# Autodesk Inventor assembly: ASSEMBLY_Main
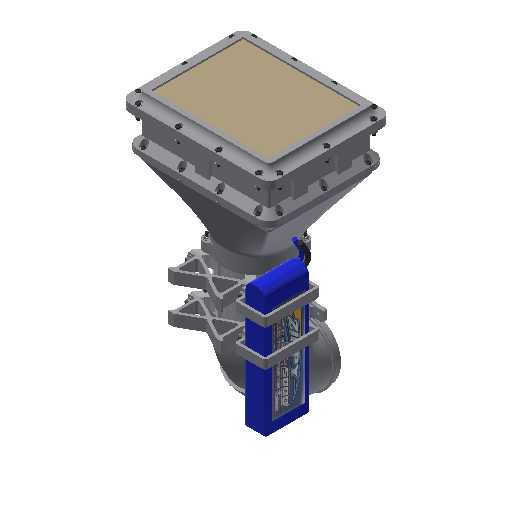
[picture p0: Inventor's stored thumbnail of the model, 512x512]
Saved by Autodesk Inventor 2025 (Build 290162010, 162A)
## iProperties
Created: 2020-03-28
Part Number: ASSEMBLY_Main
Document SubType Name: Assembly
Designer: Andrzej
Author: Andrzej
## Documents named in this file (25)
- D:\_ANDRZEJ_LACZEWSKI\_OTHER\MECH - Air Filtering Unit & Positive Pressure Suit (COVID-19)\MCAD\1_REV1\ASSEMBLY_MAIN_REVA\ASSEMBLY_Main.iam
- D:\_ANDRZEJ_LACZEWSKI\_OTHER\MECH - Air Filtering Unit & Positive Pressure Suit (COVID-19)\MCAD\1_REV1\ASSEMBLY_MAIN_REVA\3DP_PLA_Filter_stage.ipt
- D:\_ANDRZEJ_LACZEWSKI\_OTHER\MECH - Air Filtering Unit & Positive Pressure Suit (COVID-19)\MCAD\1_REV1\__COTS_PARTS\COTS_HP_BLC7000_Fan_Case.ipt
- D:\_ANDRZEJ_LACZEWSKI\_OTHER\MECH - Air Filtering Unit & Positive Pressure Suit (COVID-19)\MCAD\1_REV1\__COTS_PARTS\COTS_Zelmer_108x137mm_HEPA_filter.ipt
- D:\_ANDRZEJ_LACZEWSKI\_OTHER\MECH - Air Filtering Unit & Positive Pressure Suit (COVID-19)\MCAD\1_REV1\ASSEMBLY_MAIN_REVA\3DP_PLA_Filter_stage_to_turbine_adapter.ipt
- D:\_ANDRZEJ_LACZEWSKI\_OTHER\MECH - Air Filtering Unit & Positive Pressure Suit (COVID-19)\MCAD\1_REV1\ASSEMBLY_MAIN_REVA\3DP_PLA_Turbine_stand.ipt
- D:\_ANDRZEJ_LACZEWSKI\_OTHER\MECH - Air Filtering Unit & Positive Pressure Suit (COVID-19)\MCAD\1_REV1\ASSEMBLY_MAIN_REVA\3DP_PLA_Internal_filter_mesh.ipt
- D:\_ANDRZEJ_LACZEWSKI\_OTHER\MECH - Air Filtering Unit & Positive Pressure Suit (COVID-19)\MCAD\1_REV1\ASSEMBLY_MAIN_REVA\3DP_PLA_Front_filter_mount_hood.ipt
- D:\_ANDRZEJ_LACZEWSKI\_OTHER\MECH - Air Filtering Unit & Positive Pressure Suit (COVID-19)\MCAD\1_REV1\ASSEMBLY_MAIN_REVA\3DP_PLA_Front_filter_mount_hood_spacer.ipt
- D:\_ANDRZEJ_LACZEWSKI\_OTHER\MECH - Air Filtering Unit & Positive Pressure Suit (COVID-19)\MCAD\1_REV1\ASSEMBLY_MAIN_REVA\3DP_PLA_Front_filter_mesh.ipt
- D:\_ANDRZEJ_LACZEWSKI\_OTHER\MECH - Air Filtering Unit & Positive Pressure Suit (COVID-19)\MCAD\1_REV1\__COTS_PARTS\COTS_ZIPPY_Li-Po_Battery_5000mAh_3S.ipt
- D:\_ANDRZEJ_LACZEWSKI\_OTHER\MECH - Air Filtering Unit & Positive Pressure Suit (COVID-19)\MCAD\1_REV1\ASSEMBLY_MAIN_REVA\3DP_PLA_Battery_mount.ipt
- D:\_ANDRZEJ_LACZEWSKI\_OTHER\MECH - Air Filtering Unit & Positive Pressure Suit (COVID-19)\MCAD\1_REV1\ASSEMBLY_MAIN_REVA\3DP_PLA_Turbine_exhaust_bottom_part.ipt
- D:\_ANDRZEJ_LACZEWSKI\_OTHER\MECH - Air Filtering Unit & Positive Pressure Suit (COVID-19)\MCAD\1_REV1\ASSEMBLY_MAIN_REVA\3DP_PLA_Turbine_exhaust_top_part.ipt
- D:\_ANDRZEJ_LACZEWSKI\_OTHER\MECH - Air Filtering Unit & Positive Pressure Suit (COVID-19)\MCAD\1_REV1\ASSEMBLY_MAIN_REVA\3DP_PLA_Switch_&_handle_mount_plate.ipt
- D:\_ANDRZEJ_LACZEWSKI\_OTHER\MECH - Air Filtering Unit & Positive Pressure Suit (COVID-19)\MCAD\1_REV1\__CONTENT_CENTER_PARTS\en-US\DIN 125-2  A\DIN 125-2 - A 3,2A.ipt
- D:\_ANDRZEJ_LACZEWSKI\_OTHER\MECH - Air Filtering Unit & Positive Pressure Suit (COVID-19)\MCAD\1_REV1\__CONTENT_CENTER_PARTS\en-US\ISO 7380-1\ISO 7380-1 - M3 x 16.ipt
- D:\_ANDRZEJ_LACZEWSKI\_OTHER\MECH - Air Filtering Unit & Positive Pressure Suit (COVID-19)\MCAD\1_REV1\__CONTENT_CENTER_PARTS\en-US\DIN 934\DIN 934 - M3 x 0,5.ipt
- D:\_ANDRZEJ_LACZEWSKI\_OTHER\MECH - Air Filtering Unit & Positive Pressure Suit (COVID-19)\MCAD\1_REV1\__CONTENT_CENTER_PARTS\en-US\ISO 7380-1\ISO 7380-1 - M3 x 10.ipt
- D:\_ANDRZEJ_LACZEWSKI\_OTHER\MECH - Air Filtering Unit & Positive Pressure Suit (COVID-19)\MCAD\1_REV1\__CONTENT_CENTER_PARTS\en-US\DIN 125-2  A\DIN 125-2 - A 4,3A.ipt
- D:\_ANDRZEJ_LACZEWSKI\_OTHER\MECH - Air Filtering Unit & Positive Pressure Suit (COVID-19)\MCAD\1_REV1\__CONTENT_CENTER_PARTS\en-US\ISO 7380-1\ISO 7380-1 - M4 x 12.ipt
- D:\_ANDRZEJ_LACZEWSKI\_OTHER\MECH - Air Filtering Unit & Positive Pressure Suit (COVID-19)\MCAD\1_REV1\__CONTENT_CENTER_PARTS\en-US\DIN 934\DIN 934 - M4 x 0,7.ipt
- D:\_ANDRZEJ_LACZEWSKI\_OTHER\MECH - Air Filtering Unit & Positive Pressure Suit (COVID-19)\MCAD\1_REV1\__CONTENT_CENTER_PARTS\en-US\ISO 7380-1\ISO 7380-1 - M3 x 30.ipt
- D:\_ANDRZEJ_LACZEWSKI\_OTHER\MECH - Air Filtering Unit & Positive Pressure Suit (COVID-19)\MCAD\1_REV1\__CONTENT_CENTER_PARTS\en-US\ISO 7380-1\ISO 7380-1 - M4 x 20.ipt
- D:\_ANDRZEJ_LACZEWSKI\_OTHER\MECH - Air Filtering Unit & Positive Pressure Suit (COVID-19)\MCAD\1_REV1\__CONTENT_CENTER_PARTS\en-US\ISO 7380-1\ISO 7380-1 - M4 x 16.ipt
## Components (164 placed, 24 different names)
1. 3DP_PLA_Filter_stage:1 — Mate:1, Mate:2, Mate:3, Mate:4, Flush:1, Flush:2, Mate:13, Mate:14, Mate:16, Flush:3, Flush:4, Mate:82, Mate:84, Mate:86, Mate:88, Mate:90, Mate:92, Mate:94, Mate:96, Mate:98, Mate:100, Mate:102, Mate:104, Mate:106, Mate:108, Mate:109, Mate:110, Mate:111, Mate:112, Mate:113, Mate:114, Mate:115, Mate:116, Mate:117, Mate:118, Mate:119, Mate:120, Mate:121, Mate:122, Mate:123, Mate:124, Mate:125, Mate:126, Mate:127, Mate:128, Mate:129, Mate:130, Mate:131, Mate:132, Mate:133, Mate:134, Mate:135, Mate:136, Mate:137, Mate:139, Mate:141, Mate:143, Mate:145, Mate:147, Mate:149, Mate:151, Mate:153, Mate:155, Mate:157, Mate:159, Mate:161, Mate:163
2. COTS_HP_BLC7000_Fan_Case:1 — Mate:5, Mate:6, Mate:9, Mate:10, Mate:11, Mate:21, Mate:22, Mate:26, Mate:27, Mate:28, Mate:29, Mate:30, Mate:31, Mate:32, Mate:33, Mate:48, Mate:49, Mate:50, Mate:165, Mate:166, Mate:167, Mate:168, Mate:169, Mate:171, Mate:173, Mate:174, Mate:175, Mate:176, Mate:177, Mate:179, Mate:181, Mate:182, Mate:183, Mate:184, Mate:185, Mate:187
3. COTS_Zelmer_108x137mm_HEPA_filter:1 — Mate:1, Mate:2, Mate:3, Mate:23
4. 3DP_PLA_Filter_stage_to_turbine_adapter:1 — Mate:4, Flush:1, Flush:2, Mate:5, Mate:6, Mate:9, Mate:12, Mate:138, Mate:140, Mate:142, Mate:144, Mate:146, Mate:148, Mate:150, Mate:152, Mate:154, Mate:156, Mate:158, Mate:160, Mate:162, Mate:164, Mate:178, Mate:180
5. 3DP_PLA_Turbine_stand:1 — Mate:10, Mate:11, Mate:26
6. 3DP_PLA_Internal_filter_mesh:1 — Mate:12, Mate:13, Mate:14
7. 3DP_PLA_Front_filter_mount_hood:1 — Mate:17, Flush:5, Flush:6, Mate:44, Mate:45, Mate:53, Mate:54, Mate:55, Mate:56, Mate:57, Mate:58, Mate:59, Mate:60, Mate:61, Mate:62, Mate:63, Mate:64, Mate:65, Mate:66, Mate:67, Mate:68, Mate:69, Mate:70, Mate:71, Mate:72, Mate:73, Mate:74, Mate:75, Mate:76, Mate:77, Mate:78, Mate:79, Mate:80, Mate:81, Mate:83, Mate:85, Mate:87, Mate:89, Mate:91, Mate:93, Mate:95, Mate:97, Mate:99, Mate:101, Mate:103, Mate:105, Mate:107
8. 3DP_PLA_Front_filter_mount_hood_spacer:1 — Mate:16, Flush:3, Flush:4, Mate:17, Flush:5, Flush:6
9. 3DP_PLA_Turbine_stand:2 — Mate:21, Mate:22, Mate:27, Mate:170, Mate:172
10. 3DP_PLA_Front_filter_mesh:1 — Mate:23, Mate:44, Mate:45
11. COTS_ZIPPY_Li-Po_Battery_5000mAh_3S:1 — Mate:34, Mate:35
12. 3DP_PLA_Battery_mount:1 — Mate:28, Mate:29, Mate:30, Mate:34, Mate:35, Mate:189, Mate:190, Mate:192, Mate:193, Mate:194, Mate:196
13. 3DP_PLA_Battery_mount:2 — Mate:31, Mate:32, Mate:33, Mate:191, Mate:195
14. 3DP_PLA_Turbine_exhaust_bottom_part:1 — Mate:46, Mate:47, Tangent:1, Mate:48, Mate:49, Mate:50, Mate:51, Mate:52, Mate:186, Mate:188
15. 3DP_PLA_Turbine_exhaust_top_part:1 — Mate:46, Mate:47, Tangent:1
16. 3DP_PLA_Switch_&_handle_mount_plate:1 — Mate:51, Mate:52, Mate:197, Mate:198, Mate:199, Mate:200
17. ISO 7380-1 M4 x 16:2 — Insert:74
18. DIN 125-2 A A 4,3:10 — Mate:199, Mate:200, Insert:74
19. ISO 7380-1 M4 x 16:1 — Insert:73
20. DIN 125-2 A A 4,3:9 — Mate:197, Mate:198, Insert:73
21. DIN 934 - replaced by DIN EN 24032/28673/28674 M4:4 — Insert:72
22. DIN 125-2 A A 4,3:8 — Mate:195, Mate:196, Insert:72
23. ISO 7380-1 M4 x 20:2 — Insert:70
24. DIN 125-2 A A 4,3:7 — Mate:191, Mate:192, Insert:70
25. DIN 934 - replaced by DIN EN 24032/28673/28674 M4:3 — Insert:71
26. DIN 125-2 A A 4,3:6 — Mate:193, Mate:194, Insert:71
27. ISO 7380-1 M4 x 20:1 — Insert:69
28. DIN 125-2 A A 4,3:5 — Mate:189, Mate:190, Insert:69
29. DIN 934 - replaced by DIN EN 24032/28673/28674 M3:32 — Insert:68
30. DIN 125-2 A A 3,2:64 — Mate:187, Mate:188, Insert:68
31. ISO 7380-1 M3 x 30:4 — Insert:66
32. DIN 125-2 A A 3,2:63 — Mate:183, Mate:184, Insert:66
33. DIN 934 - replaced by DIN EN 24032/28673/28674 M3:31 — Insert:67
34. DIN 125-2 A A 3,2:62 — Mate:185, Mate:186, Insert:67
35. ISO 7380-1 M3 x 30:3 — Insert:65
36. DIN 125-2 A A 3,2:61 — Mate:181, Mate:182, Insert:65
37. DIN 934 - replaced by DIN EN 24032/28673/28674 M3:30 — Insert:64
38. DIN 125-2 A A 3,2:60 — Mate:179, Mate:180, Insert:64
39. ISO 7380-1 M3 x 30:2 — Insert:62
40. DIN 125-2 A A 3,2:59 — Mate:175, Mate:176, Insert:62
41. DIN 934 - replaced by DIN EN 24032/28673/28674 M3:29 — Insert:63
42. DIN 125-2 A A 3,2:58 — Mate:177, Mate:178, Insert:63
43. ISO 7380-1 M3 x 30:1 — Insert:61
44. DIN 125-2 A A 3,2:57 — Mate:173, Mate:174, Insert:61
45. DIN 934 - replaced by DIN EN 24032/28673/28674 M4:2 — Insert:60
46. DIN 125-2 A A 4,3:4 — Mate:171, Mate:172, Insert:60
47. ISO 7380-1 M4 x 12:2 — Insert:58
48. DIN 125-2 A A 4,3:3 — Mate:167, Mate:168, Insert:58
49. DIN 934 - replaced by DIN EN 24032/28673/28674 M4:1 — Insert:59
50. DIN 125-2 A A 4,3:2 — Mate:169, Mate:170, Insert:59
51. ISO 7380-1 M4 x 12:1 — Insert:57
52. DIN 125-2 A A 4,3:1 — Mate:165, Mate:166, Insert:57
53. DIN 934 - replaced by DIN EN 24032/28673/28674 M3:28 — Insert:56
54. DIN 934 - replaced by DIN EN 24032/28673/28674 M3:27 — Insert:55
55. DIN 934 - replaced by DIN EN 24032/28673/28674 M3:26 — Insert:54
56. DIN 934 - replaced by DIN EN 24032/28673/28674 M3:25 — Insert:53
57. DIN 934 - replaced by DIN EN 24032/28673/28674 M3:24 — Insert:52
58. DIN 934 - replaced by DIN EN 24032/28673/28674 M3:23 — Insert:51
59. DIN 934 - replaced by DIN EN 24032/28673/28674 M3:22 — Insert:50
60. DIN 934 - replaced by DIN EN 24032/28673/28674 M3:21 — Insert:49
61. DIN 934 - replaced by DIN EN 24032/28673/28674 M3:20 — Insert:48
62. DIN 934 - replaced by DIN EN 24032/28673/28674 M3:19 — Insert:47
63. DIN 934 - replaced by DIN EN 24032/28673/28674 M3:18 — Insert:46
64. DIN 934 - replaced by DIN EN 24032/28673/28674 M3:17 — Insert:45
65. DIN 934 - replaced by DIN EN 24032/28673/28674 M3:16 — Insert:44
66. DIN 125-2 A A 3,2:56 — Mate:163, Mate:164, Insert:56
67. DIN 125-2 A A 3,2:55 — Mate:161, Mate:162, Insert:55
68. DIN 125-2 A A 3,2:54 — Mate:159, Mate:160, Insert:54
69. DIN 125-2 A A 3,2:53 — Mate:157, Mate:158, Insert:53
70. DIN 125-2 A A 3,2:52 — Mate:155, Mate:156, Insert:52
71. DIN 125-2 A A 3,2:51 — Mate:153, Mate:154, Insert:51
72. DIN 125-2 A A 3,2:50 — Mate:151, Mate:152, Insert:50
73. DIN 125-2 A A 3,2:49 — Mate:149, Mate:150, Insert:49
74. DIN 125-2 A A 3,2:48 — Mate:147, Mate:148, Insert:48
75. DIN 125-2 A A 3,2:47 — Mate:145, Mate:146, Insert:47
76. DIN 125-2 A A 3,2:46 — Mate:143, Mate:144, Insert:46
77. DIN 125-2 A A 3,2:45 — Mate:141, Mate:142, Insert:45
78. DIN 125-2 A A 3,2:44 — Mate:139, Mate:140, Insert:44
79. ISO 7380-1 M3 x 10:14 — Insert:42
80. ISO 7380-1 M3 x 10:13 — Insert:41
81. ISO 7380-1 M3 x 10:12 — Insert:40
82. ISO 7380-1 M3 x 10:11 — Insert:39
83. ISO 7380-1 M3 x 10:10 — Insert:38
84. ISO 7380-1 M3 x 10:9 — Insert:37
85. ISO 7380-1 M3 x 10:8 — Insert:36
86. ISO 7380-1 M3 x 10:7 — Insert:35
87. ISO 7380-1 M3 x 10:6 — Insert:34
88. ISO 7380-1 M3 x 10:5 — Insert:33
89. ISO 7380-1 M3 x 10:4 — Insert:32
90. ISO 7380-1 M3 x 10:3 — Insert:31
91. ISO 7380-1 M3 x 10:2 — Insert:30
92. DIN 125-2 A A 3,2:43 — Mate:135, Mate:136, Insert:42
93. DIN 125-2 A A 3,2:42 — Mate:133, Mate:134, Insert:41
94. DIN 125-2 A A 3,2:41 — Mate:131, Mate:132, Insert:40
95. DIN 125-2 A A 3,2:40 — Mate:129, Mate:130, Insert:39
96. DIN 125-2 A A 3,2:39 — Mate:127, Mate:128, Insert:38
97. DIN 125-2 A A 3,2:38 — Mate:125, Mate:126, Insert:37
98. DIN 125-2 A A 3,2:37 — Mate:123, Mate:124, Insert:36
99. DIN 125-2 A A 3,2:36 — Mate:121, Mate:122, Insert:35
100. DIN 125-2 A A 3,2:35 — Mate:119, Mate:120, Insert:34
101. DIN 125-2 A A 3,2:34 — Mate:117, Mate:118, Insert:33
102. DIN 125-2 A A 3,2:33 — Mate:115, Mate:116, Insert:32
103. DIN 125-2 A A 3,2:32 — Mate:113, Mate:114, Insert:31
104. DIN 125-2 A A 3,2:31 — Mate:111, Mate:112, Insert:30
105. DIN 934 - replaced by DIN EN 24032/28673/28674 M3:15 — Insert:43
106. DIN 125-2 A A 3,2:30 — Mate:137, Mate:138, Insert:43
107. ISO 7380-1 M3 x 10:1 — Insert:29
108. DIN 125-2 A A 3,2:29 — Mate:109, Mate:110, Insert:29
109. DIN 934 - replaced by DIN EN 24032/28673/28674 M3:14 — Insert:28
110. DIN 934 - replaced by DIN EN 24032/28673/28674 M3:13 — Insert:27
111. DIN 934 - replaced by DIN EN 24032/28673/28674 M3:12 — Insert:26
112. DIN 934 - replaced by DIN EN 24032/28673/28674 M3:11 — Insert:25
113. DIN 934 - replaced by DIN EN 24032/28673/28674 M3:10 — Insert:24
114. DIN 934 - replaced by DIN EN 24032/28673/28674 M3:9 — Insert:23
115. DIN 934 - replaced by DIN EN 24032/28673/28674 M3:8 — Insert:22
116. DIN 934 - replaced by DIN EN 24032/28673/28674 M3:7 — Insert:21
117. DIN 934 - replaced by DIN EN 24032/28673/28674 M3:6 — Insert:20
118. DIN 934 - replaced by DIN EN 24032/28673/28674 M3:5 — Insert:19
119. DIN 934 - replaced by DIN EN 24032/28673/28674 M3:4 — Insert:18
120. DIN 934 - replaced by DIN EN 24032/28673/28674 M3:3 — Insert:17
121. DIN 934 - replaced by DIN EN 24032/28673/28674 M3:2 — Insert:16
122. DIN 125-2 A A 3,2:28 — Mate:107, Mate:108, Insert:28
123. DIN 125-2 A A 3,2:27 — Mate:105, Mate:106, Insert:27
124. DIN 125-2 A A 3,2:26 — Mate:103, Mate:104, Insert:26
125. DIN 125-2 A A 3,2:25 — Mate:101, Mate:102, Insert:25
126. DIN 125-2 A A 3,2:24 — Mate:99, Mate:100, Insert:24
127. DIN 125-2 A A 3,2:23 — Mate:97, Mate:98, Insert:23
128. DIN 125-2 A A 3,2:22 — Mate:95, Mate:96, Insert:22
129. DIN 125-2 A A 3,2:21 — Mate:93, Mate:94, Insert:21
130. DIN 125-2 A A 3,2:20 — Mate:91, Mate:92, Insert:20
131. DIN 125-2 A A 3,2:19 — Mate:89, Mate:90, Insert:19
132. DIN 125-2 A A 3,2:18 — Mate:87, Mate:88, Insert:18
133. DIN 125-2 A A 3,2:17 — Mate:85, Mate:86, Insert:17
134. DIN 125-2 A A 3,2:16 — Mate:83, Mate:84, Insert:16
135. ISO 7380-1 M3 x 16:14 — Insert:14
136. ISO 7380-1 M3 x 16:13 — Insert:13
137. ISO 7380-1 M3 x 16:12 — Insert:12
138. ISO 7380-1 M3 x 16:11 — Insert:11
139. ISO 7380-1 M3 x 16:10 — Insert:10
140. ISO 7380-1 M3 x 16:9 — Insert:9
141. ISO 7380-1 M3 x 16:8 — Insert:8
142. ISO 7380-1 M3 x 16:7 — Insert:7
143. ISO 7380-1 M3 x 16:6 — Insert:6
144. ISO 7380-1 M3 x 16:5 — Insert:5
145. ISO 7380-1 M3 x 16:4 — Insert:4
146. ISO 7380-1 M3 x 16:3 — Insert:3
147. ISO 7380-1 M3 x 16:2 — Insert:2
148. DIN 125-2 A A 3,2:15 — Mate:79, Mate:80, Insert:14
149. DIN 125-2 A A 3,2:14 — Mate:77, Mate:78, Insert:13
150. DIN 125-2 A A 3,2:13 — Mate:75, Mate:76, Insert:12
151. DIN 125-2 A A 3,2:12 — Mate:73, Mate:74, Insert:11
152. DIN 125-2 A A 3,2:11 — Mate:71, Mate:72, Insert:10
153. DIN 125-2 A A 3,2:10 — Mate:69, Mate:70, Insert:9
154. DIN 125-2 A A 3,2:9 — Mate:67, Mate:68, Insert:8
155. DIN 125-2 A A 3,2:8 — Mate:65, Mate:66, Insert:7
156. DIN 125-2 A A 3,2:7 — Mate:63, Mate:64, Insert:6
157. DIN 125-2 A A 3,2:6 — Mate:61, Mate:62, Insert:5
158. DIN 125-2 A A 3,2:5 — Mate:59, Mate:60, Insert:4
159. DIN 125-2 A A 3,2:4 — Mate:57, Mate:58, Insert:3
160. DIN 125-2 A A 3,2:3 — Mate:55, Mate:56, Insert:2
161. DIN 934 - replaced by DIN EN 24032/28673/28674 M3:1 — Insert:15
162. DIN 125-2 A A 3,2:2 — Mate:81, Mate:82, Insert:15
163. ISO 7380-1 M3 x 16:1 — Insert:1
164. DIN 125-2 A A 3,2:1 — Mate:53, Mate:54, Insert:1
## Relationships (265: Mate 184, Insert 74, Flush 6, Tangent 1)
- Mate:1: 3DP_PLA_Filter_stage:1 ↔ COTS_Zelmer_108x137mm_HEPA_filter:1
- Mate:2 (1 mm): 3DP_PLA_Filter_stage:1 ↔ COTS_Zelmer_108x137mm_HEPA_filter:1
- Mate:3 (1 mm): 3DP_PLA_Filter_stage:1 ↔ COTS_Zelmer_108x137mm_HEPA_filter:1
- Mate:4: 3DP_PLA_Filter_stage:1 ↔ 3DP_PLA_Filter_stage_to_turbine_adapter:1
- Flush:1: 3DP_PLA_Filter_stage:1 ↔ 3DP_PLA_Filter_stage_to_turbine_adapter:1
- Flush:2: 3DP_PLA_Filter_stage:1 ↔ 3DP_PLA_Filter_stage_to_turbine_adapter:1
- Mate:5: COTS_HP_BLC7000_Fan_Case:1 ↔ 3DP_PLA_Filter_stage_to_turbine_adapter:1
- Mate:6: COTS_HP_BLC7000_Fan_Case:1 ↔ 3DP_PLA_Filter_stage_to_turbine_adapter:1
- Mate:9: COTS_HP_BLC7000_Fan_Case:1 ↔ 3DP_PLA_Filter_stage_to_turbine_adapter:1
- Mate:10: COTS_HP_BLC7000_Fan_Case:1 ↔ 3DP_PLA_Turbine_stand:1
- Mate:11: COTS_HP_BLC7000_Fan_Case:1 ↔ 3DP_PLA_Turbine_stand:1
- Mate:12: 3DP_PLA_Filter_stage_to_turbine_adapter:1 ↔ 3DP_PLA_Internal_filter_mesh:1
- Mate:13 (0.5 mm): 3DP_PLA_Filter_stage:1 ↔ 3DP_PLA_Internal_filter_mesh:1
- Mate:14 (0.5 mm): 3DP_PLA_Filter_stage:1 ↔ 3DP_PLA_Internal_filter_mesh:1
- Mate:16: 3DP_PLA_Filter_stage:1 ↔ 3DP_PLA_Front_filter_mount_hood_spacer:1
- Flush:3: 3DP_PLA_Filter_stage:1 ↔ 3DP_PLA_Front_filter_mount_hood_spacer:1
- Flush:4: 3DP_PLA_Filter_stage:1 ↔ 3DP_PLA_Front_filter_mount_hood_spacer:1
- Mate:17: 3DP_PLA_Front_filter_mount_hood:1 ↔ 3DP_PLA_Front_filter_mount_hood_spacer:1
- Flush:5: 3DP_PLA_Front_filter_mount_hood:1 ↔ 3DP_PLA_Front_filter_mount_hood_spacer:1
- Flush:6: 3DP_PLA_Front_filter_mount_hood:1 ↔ 3DP_PLA_Front_filter_mount_hood_spacer:1
- Mate:21: COTS_HP_BLC7000_Fan_Case:1 ↔ 3DP_PLA_Turbine_stand:2
- Mate:22: COTS_HP_BLC7000_Fan_Case:1 ↔ 3DP_PLA_Turbine_stand:2
- Mate:23 (3 mm): COTS_Zelmer_108x137mm_HEPA_filter:1 ↔ 3DP_PLA_Front_filter_mesh:1
- Mate:26: COTS_HP_BLC7000_Fan_Case:1 ↔ 3DP_PLA_Turbine_stand:1
- Mate:27: COTS_HP_BLC7000_Fan_Case:1 ↔ 3DP_PLA_Turbine_stand:2
- Mate:28 (0.1 mm): COTS_HP_BLC7000_Fan_Case:1 ↔ 3DP_PLA_Battery_mount:1
- Mate:29: COTS_HP_BLC7000_Fan_Case:1 ↔ 3DP_PLA_Battery_mount:1
- Mate:30: COTS_HP_BLC7000_Fan_Case:1 ↔ 3DP_PLA_Battery_mount:1
- Mate:31: COTS_HP_BLC7000_Fan_Case:1 ↔ 3DP_PLA_Battery_mount:2
- Mate:32 (0.1 mm): COTS_HP_BLC7000_Fan_Case:1 ↔ 3DP_PLA_Battery_mount:2
- Mate:33: COTS_HP_BLC7000_Fan_Case:1 ↔ 3DP_PLA_Battery_mount:2
- Mate:34 (3 mm): COTS_ZIPPY_Li-Po_Battery_5000mAh_3S:1 ↔ 3DP_PLA_Battery_mount:1
- Mate:35 (3 mm): COTS_ZIPPY_Li-Po_Battery_5000mAh_3S:1 ↔ 3DP_PLA_Battery_mount:1
- Mate:44 (0.5 mm): 3DP_PLA_Front_filter_mount_hood:1 ↔ 3DP_PLA_Front_filter_mesh:1
- Mate:45 (0.5 mm): 3DP_PLA_Front_filter_mount_hood:1 ↔ 3DP_PLA_Front_filter_mesh:1
- Mate:46: 3DP_PLA_Turbine_exhaust_bottom_part:1 ↔ 3DP_PLA_Turbine_exhaust_top_part:1
- Mate:47: 3DP_PLA_Turbine_exhaust_bottom_part:1 ↔ 3DP_PLA_Turbine_exhaust_top_part:1
- Tangent:1: 3DP_PLA_Turbine_exhaust_bottom_part:1 ↔ 3DP_PLA_Turbine_exhaust_top_part:1
- Mate:48: COTS_HP_BLC7000_Fan_Case:1 ↔ 3DP_PLA_Turbine_exhaust_bottom_part:1
- Mate:49: COTS_HP_BLC7000_Fan_Case:1 ↔ 3DP_PLA_Turbine_exhaust_bottom_part:1
- Mate:50: COTS_HP_BLC7000_Fan_Case:1 ↔ 3DP_PLA_Turbine_exhaust_bottom_part:1
- Mate:51: 3DP_PLA_Turbine_exhaust_bottom_part:1 ↔ 3DP_PLA_Switch_&_handle_mount_plate:1
- Mate:52: 3DP_PLA_Turbine_exhaust_bottom_part:1 ↔ 3DP_PLA_Switch_&_handle_mount_plate:1
- Mate:53: 3DP_PLA_Front_filter_mount_hood:1 ↔ DIN 125-2 A A 3,2:1
- Mate:54: 3DP_PLA_Front_filter_mount_hood:1 ↔ DIN 125-2 A A 3,2:1
- Mate:55: 3DP_PLA_Front_filter_mount_hood:1 ↔ DIN 125-2 A A 3,2:3
- Mate:56: 3DP_PLA_Front_filter_mount_hood:1 ↔ DIN 125-2 A A 3,2:3
- Mate:57: 3DP_PLA_Front_filter_mount_hood:1 ↔ DIN 125-2 A A 3,2:4
- Mate:58: 3DP_PLA_Front_filter_mount_hood:1 ↔ DIN 125-2 A A 3,2:4
- Mate:59: 3DP_PLA_Front_filter_mount_hood:1 ↔ DIN 125-2 A A 3,2:5
- Mate:60: 3DP_PLA_Front_filter_mount_hood:1 ↔ DIN 125-2 A A 3,2:5
- Mate:61: 3DP_PLA_Front_filter_mount_hood:1 ↔ DIN 125-2 A A 3,2:6
- Mate:62: 3DP_PLA_Front_filter_mount_hood:1 ↔ DIN 125-2 A A 3,2:6
- Mate:63: 3DP_PLA_Front_filter_mount_hood:1 ↔ DIN 125-2 A A 3,2:7
- Mate:64: 3DP_PLA_Front_filter_mount_hood:1 ↔ DIN 125-2 A A 3,2:7
- Mate:65: 3DP_PLA_Front_filter_mount_hood:1 ↔ DIN 125-2 A A 3,2:8
- Mate:66: 3DP_PLA_Front_filter_mount_hood:1 ↔ DIN 125-2 A A 3,2:8
- Mate:67: 3DP_PLA_Front_filter_mount_hood:1 ↔ DIN 125-2 A A 3,2:9
- Mate:68: 3DP_PLA_Front_filter_mount_hood:1 ↔ DIN 125-2 A A 3,2:9
- Mate:69: 3DP_PLA_Front_filter_mount_hood:1 ↔ DIN 125-2 A A 3,2:10
- Mate:70: 3DP_PLA_Front_filter_mount_hood:1 ↔ DIN 125-2 A A 3,2:10
- Mate:71: 3DP_PLA_Front_filter_mount_hood:1 ↔ DIN 125-2 A A 3,2:11
- Mate:72: 3DP_PLA_Front_filter_mount_hood:1 ↔ DIN 125-2 A A 3,2:11
- Mate:73: 3DP_PLA_Front_filter_mount_hood:1 ↔ DIN 125-2 A A 3,2:12
- Mate:74: 3DP_PLA_Front_filter_mount_hood:1 ↔ DIN 125-2 A A 3,2:12
- Mate:75: 3DP_PLA_Front_filter_mount_hood:1 ↔ DIN 125-2 A A 3,2:13
- Mate:76: 3DP_PLA_Front_filter_mount_hood:1 ↔ DIN 125-2 A A 3,2:13
- Mate:77: 3DP_PLA_Front_filter_mount_hood:1 ↔ DIN 125-2 A A 3,2:14
- Mate:78: 3DP_PLA_Front_filter_mount_hood:1 ↔ DIN 125-2 A A 3,2:14
- Mate:79: 3DP_PLA_Front_filter_mount_hood:1 ↔ DIN 125-2 A A 3,2:15
- Mate:80: 3DP_PLA_Front_filter_mount_hood:1 ↔ DIN 125-2 A A 3,2:15
- Insert:1: ISO 7380-1 M3 x 16:1 ↔ DIN 125-2 A A 3,2:1
- Insert:2: ISO 7380-1 M3 x 16:2 ↔ DIN 125-2 A A 3,2:3
- Insert:3: ISO 7380-1 M3 x 16:3 ↔ DIN 125-2 A A 3,2:4
- Insert:4: ISO 7380-1 M3 x 16:4 ↔ DIN 125-2 A A 3,2:5
- Insert:5: ISO 7380-1 M3 x 16:5 ↔ DIN 125-2 A A 3,2:6
- Insert:6: ISO 7380-1 M3 x 16:6 ↔ DIN 125-2 A A 3,2:7
- Insert:7: ISO 7380-1 M3 x 16:7 ↔ DIN 125-2 A A 3,2:8
- Insert:8: ISO 7380-1 M3 x 16:8 ↔ DIN 125-2 A A 3,2:9
- Insert:9: ISO 7380-1 M3 x 16:9 ↔ DIN 125-2 A A 3,2:10
- Insert:10: ISO 7380-1 M3 x 16:10 ↔ DIN 125-2 A A 3,2:11
- Insert:11: ISO 7380-1 M3 x 16:11 ↔ DIN 125-2 A A 3,2:12
- Insert:12: ISO 7380-1 M3 x 16:12 ↔ DIN 125-2 A A 3,2:13
- Insert:13: ISO 7380-1 M3 x 16:13 ↔ DIN 125-2 A A 3,2:14
- Insert:14: ISO 7380-1 M3 x 16:14 ↔ DIN 125-2 A A 3,2:15
- Mate:81: 3DP_PLA_Front_filter_mount_hood:1 ↔ DIN 125-2 A A 3,2:2
- Mate:82: 3DP_PLA_Filter_stage:1 ↔ DIN 125-2 A A 3,2:2
- Mate:83: 3DP_PLA_Front_filter_mount_hood:1 ↔ DIN 125-2 A A 3,2:16
- Mate:84: 3DP_PLA_Filter_stage:1 ↔ DIN 125-2 A A 3,2:16
- Mate:85: 3DP_PLA_Front_filter_mount_hood:1 ↔ DIN 125-2 A A 3,2:17
- Mate:86: 3DP_PLA_Filter_stage:1 ↔ DIN 125-2 A A 3,2:17
- Mate:87: 3DP_PLA_Front_filter_mount_hood:1 ↔ DIN 125-2 A A 3,2:18
- Mate:88: 3DP_PLA_Filter_stage:1 ↔ DIN 125-2 A A 3,2:18
- Mate:89: 3DP_PLA_Front_filter_mount_hood:1 ↔ DIN 125-2 A A 3,2:19
- Mate:90: 3DP_PLA_Filter_stage:1 ↔ DIN 125-2 A A 3,2:19
- Mate:91: 3DP_PLA_Front_filter_mount_hood:1 ↔ DIN 125-2 A A 3,2:20
- Mate:92: 3DP_PLA_Filter_stage:1 ↔ DIN 125-2 A A 3,2:20
- Mate:93: 3DP_PLA_Front_filter_mount_hood:1 ↔ DIN 125-2 A A 3,2:21
- Mate:94: 3DP_PLA_Filter_stage:1 ↔ DIN 125-2 A A 3,2:21
- Mate:95: 3DP_PLA_Front_filter_mount_hood:1 ↔ DIN 125-2 A A 3,2:22
- Mate:96: 3DP_PLA_Filter_stage:1 ↔ DIN 125-2 A A 3,2:22
- Mate:97: 3DP_PLA_Front_filter_mount_hood:1 ↔ DIN 125-2 A A 3,2:23
- Mate:98: 3DP_PLA_Filter_stage:1 ↔ DIN 125-2 A A 3,2:23
- Mate:99: 3DP_PLA_Front_filter_mount_hood:1 ↔ DIN 125-2 A A 3,2:24
- Mate:100: 3DP_PLA_Filter_stage:1 ↔ DIN 125-2 A A 3,2:24
- Mate:101: 3DP_PLA_Front_filter_mount_hood:1 ↔ DIN 125-2 A A 3,2:25
- Mate:102: 3DP_PLA_Filter_stage:1 ↔ DIN 125-2 A A 3,2:25
- Mate:103: 3DP_PLA_Front_filter_mount_hood:1 ↔ DIN 125-2 A A 3,2:26
- Mate:104: 3DP_PLA_Filter_stage:1 ↔ DIN 125-2 A A 3,2:26
- Mate:105: 3DP_PLA_Front_filter_mount_hood:1 ↔ DIN 125-2 A A 3,2:27
- Mate:106: 3DP_PLA_Filter_stage:1 ↔ DIN 125-2 A A 3,2:27
- Mate:107: 3DP_PLA_Front_filter_mount_hood:1 ↔ DIN 125-2 A A 3,2:28
- Mate:108: 3DP_PLA_Filter_stage:1 ↔ DIN 125-2 A A 3,2:28
- Insert:15: DIN 934 - replaced by DIN EN 24032/28673/28674 M3:1 ↔ DIN 125-2 A A 3,2:2
- Insert:16: DIN 934 - replaced by DIN EN 24032/28673/28674 M3:2 ↔ DIN 125-2 A A 3,2:16
- Insert:17: DIN 934 - replaced by DIN EN 24032/28673/28674 M3:3 ↔ DIN 125-2 A A 3,2:17
- Insert:18: DIN 934 - replaced by DIN EN 24032/28673/28674 M3:4 ↔ DIN 125-2 A A 3,2:18
- Insert:19: DIN 934 - replaced by DIN EN 24032/28673/28674 M3:5 ↔ DIN 125-2 A A 3,2:19
- Insert:20: DIN 934 - replaced by DIN EN 24032/28673/28674 M3:6 ↔ DIN 125-2 A A 3,2:20
- Insert:21: DIN 934 - replaced by DIN EN 24032/28673/28674 M3:7 ↔ DIN 125-2 A A 3,2:21
- Insert:22: DIN 934 - replaced by DIN EN 24032/28673/28674 M3:8 ↔ DIN 125-2 A A 3,2:22
- Insert:23: DIN 934 - replaced by DIN EN 24032/28673/28674 M3:9 ↔ DIN 125-2 A A 3,2:23
- Insert:24: DIN 934 - replaced by DIN EN 24032/28673/28674 M3:10 ↔ DIN 125-2 A A 3,2:24
- Insert:25: DIN 934 - replaced by DIN EN 24032/28673/28674 M3:11 ↔ DIN 125-2 A A 3,2:25
- Insert:26: DIN 934 - replaced by DIN EN 24032/28673/28674 M3:12 ↔ DIN 125-2 A A 3,2:26
- Insert:27: DIN 934 - replaced by DIN EN 24032/28673/28674 M3:13 ↔ DIN 125-2 A A 3,2:27
- Insert:28: DIN 934 - replaced by DIN EN 24032/28673/28674 M3:14 ↔ DIN 125-2 A A 3,2:28
- Mate:109: 3DP_PLA_Filter_stage:1 ↔ DIN 125-2 A A 3,2:29
- Mate:110: 3DP_PLA_Filter_stage:1 ↔ DIN 125-2 A A 3,2:29
- Mate:111: 3DP_PLA_Filter_stage:1 ↔ DIN 125-2 A A 3,2:31
- Mate:112: 3DP_PLA_Filter_stage:1 ↔ DIN 125-2 A A 3,2:31
- Mate:113: 3DP_PLA_Filter_stage:1 ↔ DIN 125-2 A A 3,2:32
- Mate:114: 3DP_PLA_Filter_stage:1 ↔ DIN 125-2 A A 3,2:32
- Mate:115: 3DP_PLA_Filter_stage:1 ↔ DIN 125-2 A A 3,2:33
- Mate:116: 3DP_PLA_Filter_stage:1 ↔ DIN 125-2 A A 3,2:33
- Mate:117: 3DP_PLA_Filter_stage:1 ↔ DIN 125-2 A A 3,2:34
- Mate:118: 3DP_PLA_Filter_stage:1 ↔ DIN 125-2 A A 3,2:34
- Mate:119: 3DP_PLA_Filter_stage:1 ↔ DIN 125-2 A A 3,2:35
- Mate:120: 3DP_PLA_Filter_stage:1 ↔ DIN 125-2 A A 3,2:35
- Mate:121: 3DP_PLA_Filter_stage:1 ↔ DIN 125-2 A A 3,2:36
- Mate:122: 3DP_PLA_Filter_stage:1 ↔ DIN 125-2 A A 3,2:36
- Mate:123: 3DP_PLA_Filter_stage:1 ↔ DIN 125-2 A A 3,2:37
- Mate:124: 3DP_PLA_Filter_stage:1 ↔ DIN 125-2 A A 3,2:37
- Mate:125: 3DP_PLA_Filter_stage:1 ↔ DIN 125-2 A A 3,2:38
- Mate:126: 3DP_PLA_Filter_stage:1 ↔ DIN 125-2 A A 3,2:38
- Mate:127: 3DP_PLA_Filter_stage:1 ↔ DIN 125-2 A A 3,2:39
- Mate:128: 3DP_PLA_Filter_stage:1 ↔ DIN 125-2 A A 3,2:39
- Mate:129: 3DP_PLA_Filter_stage:1 ↔ DIN 125-2 A A 3,2:40
- Mate:130: 3DP_PLA_Filter_stage:1 ↔ DIN 125-2 A A 3,2:40
- Mate:131: 3DP_PLA_Filter_stage:1 ↔ DIN 125-2 A A 3,2:41
- Mate:132: 3DP_PLA_Filter_stage:1 ↔ DIN 125-2 A A 3,2:41
- Mate:133: 3DP_PLA_Filter_stage:1 ↔ DIN 125-2 A A 3,2:42
- Mate:134: 3DP_PLA_Filter_stage:1 ↔ DIN 125-2 A A 3,2:42
- Mate:135: 3DP_PLA_Filter_stage:1 ↔ DIN 125-2 A A 3,2:43
- Mate:136: 3DP_PLA_Filter_stage:1 ↔ DIN 125-2 A A 3,2:43
- Insert:29: ISO 7380-1 M3 x 10:1 ↔ DIN 125-2 A A 3,2:29
- Insert:30: ISO 7380-1 M3 x 10:2 ↔ DIN 125-2 A A 3,2:31
- Insert:31: ISO 7380-1 M3 x 10:3 ↔ DIN 125-2 A A 3,2:32
- Insert:32: ISO 7380-1 M3 x 10:4 ↔ DIN 125-2 A A 3,2:33
- Insert:33: ISO 7380-1 M3 x 10:5 ↔ DIN 125-2 A A 3,2:34
- Insert:34: ISO 7380-1 M3 x 10:6 ↔ DIN 125-2 A A 3,2:35
- Insert:35: ISO 7380-1 M3 x 10:7 ↔ DIN 125-2 A A 3,2:36
- Insert:36: ISO 7380-1 M3 x 10:8 ↔ DIN 125-2 A A 3,2:37
- Insert:37: ISO 7380-1 M3 x 10:9 ↔ DIN 125-2 A A 3,2:38
- Insert:38: ISO 7380-1 M3 x 10:10 ↔ DIN 125-2 A A 3,2:39
- Insert:39: ISO 7380-1 M3 x 10:11 ↔ DIN 125-2 A A 3,2:40
- Insert:40: ISO 7380-1 M3 x 10:12 ↔ DIN 125-2 A A 3,2:41
- Insert:41: ISO 7380-1 M3 x 10:13 ↔ DIN 125-2 A A 3,2:42
- Insert:42: ISO 7380-1 M3 x 10:14 ↔ DIN 125-2 A A 3,2:43
- Mate:137: 3DP_PLA_Filter_stage:1 ↔ DIN 125-2 A A 3,2:30
- Mate:138: 3DP_PLA_Filter_stage_to_turbine_adapter:1 ↔ DIN 125-2 A A 3,2:30
- Mate:139: 3DP_PLA_Filter_stage:1 ↔ DIN 125-2 A A 3,2:44
- Mate:140: 3DP_PLA_Filter_stage_to_turbine_adapter:1 ↔ DIN 125-2 A A 3,2:44
- Mate:141: 3DP_PLA_Filter_stage:1 ↔ DIN 125-2 A A 3,2:45
- Mate:142: 3DP_PLA_Filter_stage_to_turbine_adapter:1 ↔ DIN 125-2 A A 3,2:45
- Mate:143: 3DP_PLA_Filter_stage:1 ↔ DIN 125-2 A A 3,2:46
- Mate:144: 3DP_PLA_Filter_stage_to_turbine_adapter:1 ↔ DIN 125-2 A A 3,2:46
- Mate:145: 3DP_PLA_Filter_stage:1 ↔ DIN 125-2 A A 3,2:47
- Mate:146: 3DP_PLA_Filter_stage_to_turbine_adapter:1 ↔ DIN 125-2 A A 3,2:47
- Mate:147: 3DP_PLA_Filter_stage:1 ↔ DIN 125-2 A A 3,2:48
- Mate:148: 3DP_PLA_Filter_stage_to_turbine_adapter:1 ↔ DIN 125-2 A A 3,2:48
- Mate:149: 3DP_PLA_Filter_stage:1 ↔ DIN 125-2 A A 3,2:49
- Mate:150: 3DP_PLA_Filter_stage_to_turbine_adapter:1 ↔ DIN 125-2 A A 3,2:49
- Mate:151: 3DP_PLA_Filter_stage:1 ↔ DIN 125-2 A A 3,2:50
- Mate:152: 3DP_PLA_Filter_stage_to_turbine_adapter:1 ↔ DIN 125-2 A A 3,2:50
- Mate:153: 3DP_PLA_Filter_stage:1 ↔ DIN 125-2 A A 3,2:51
- Mate:154: 3DP_PLA_Filter_stage_to_turbine_adapter:1 ↔ DIN 125-2 A A 3,2:51
- Mate:155: 3DP_PLA_Filter_stage:1 ↔ DIN 125-2 A A 3,2:52
- Mate:156: 3DP_PLA_Filter_stage_to_turbine_adapter:1 ↔ DIN 125-2 A A 3,2:52
- Mate:157: 3DP_PLA_Filter_stage:1 ↔ DIN 125-2 A A 3,2:53
- Mate:158: 3DP_PLA_Filter_stage_to_turbine_adapter:1 ↔ DIN 125-2 A A 3,2:53
- Mate:159: 3DP_PLA_Filter_stage:1 ↔ DIN 125-2 A A 3,2:54
- Mate:160: 3DP_PLA_Filter_stage_to_turbine_adapter:1 ↔ DIN 125-2 A A 3,2:54
- Mate:161: 3DP_PLA_Filter_stage:1 ↔ DIN 125-2 A A 3,2:55
- Mate:162: 3DP_PLA_Filter_stage_to_turbine_adapter:1 ↔ DIN 125-2 A A 3,2:55
- Mate:163: 3DP_PLA_Filter_stage:1 ↔ DIN 125-2 A A 3,2:56
- Mate:164: 3DP_PLA_Filter_stage_to_turbine_adapter:1 ↔ DIN 125-2 A A 3,2:56
- Insert:43: DIN 934 - replaced by DIN EN 24032/28673/28674 M3:15 ↔ DIN 125-2 A A 3,2:30
- Insert:44: DIN 934 - replaced by DIN EN 24032/28673/28674 M3:16 ↔ DIN 125-2 A A 3,2:44
- Insert:45: DIN 934 - replaced by DIN EN 24032/28673/28674 M3:17 ↔ DIN 125-2 A A 3,2:45
- Insert:46: DIN 934 - replaced by DIN EN 24032/28673/28674 M3:18 ↔ DIN 125-2 A A 3,2:46
- Insert:47: DIN 934 - replaced by DIN EN 24032/28673/28674 M3:19 ↔ DIN 125-2 A A 3,2:47
- Insert:48: DIN 934 - replaced by DIN EN 24032/28673/28674 M3:20 ↔ DIN 125-2 A A 3,2:48
- Insert:49: DIN 934 - replaced by DIN EN 24032/28673/28674 M3:21 ↔ DIN 125-2 A A 3,2:49
- Insert:50: DIN 934 - replaced by DIN EN 24032/28673/28674 M3:22 ↔ DIN 125-2 A A 3,2:50
- Insert:51: DIN 934 - replaced by DIN EN 24032/28673/28674 M3:23 ↔ DIN 125-2 A A 3,2:51
- Insert:52: DIN 934 - replaced by DIN EN 24032/28673/28674 M3:24 ↔ DIN 125-2 A A 3,2:52
- Insert:53: DIN 934 - replaced by DIN EN 24032/28673/28674 M3:25 ↔ DIN 125-2 A A 3,2:53
- Insert:54: DIN 934 - replaced by DIN EN 24032/28673/28674 M3:26 ↔ DIN 125-2 A A 3,2:54
- Insert:55: DIN 934 - replaced by DIN EN 24032/28673/28674 M3:27 ↔ DIN 125-2 A A 3,2:55
- Insert:56: DIN 934 - replaced by DIN EN 24032/28673/28674 M3:28 ↔ DIN 125-2 A A 3,2:56
- Mate:165: COTS_HP_BLC7000_Fan_Case:1 ↔ DIN 125-2 A A 4,3:1
- Mate:166: COTS_HP_BLC7000_Fan_Case:1 ↔ DIN 125-2 A A 4,3:1
- Mate:167: COTS_HP_BLC7000_Fan_Case:1 ↔ DIN 125-2 A A 4,3:3
- Mate:168: COTS_HP_BLC7000_Fan_Case:1 ↔ DIN 125-2 A A 4,3:3
- Insert:57: ISO 7380-1 M4 x 12:1 ↔ DIN 125-2 A A 4,3:1
- Insert:58: ISO 7380-1 M4 x 12:2 ↔ DIN 125-2 A A 4,3:3
- Mate:169: COTS_HP_BLC7000_Fan_Case:1 ↔ DIN 125-2 A A 4,3:2
- Mate:170: 3DP_PLA_Turbine_stand:2 ↔ DIN 125-2 A A 4,3:2
- Mate:171: COTS_HP_BLC7000_Fan_Case:1 ↔ DIN 125-2 A A 4,3:4
- Mate:172: 3DP_PLA_Turbine_stand:2 ↔ DIN 125-2 A A 4,3:4
- Insert:59: DIN 934 - replaced by DIN EN 24032/28673/28674 M4:1 ↔ DIN 125-2 A A 4,3:2
- Insert:60: DIN 934 - replaced by DIN EN 24032/28673/28674 M4:2 ↔ DIN 125-2 A A 4,3:4
- Mate:173: COTS_HP_BLC7000_Fan_Case:1 ↔ DIN 125-2 A A 3,2:57
- Mate:174: COTS_HP_BLC7000_Fan_Case:1 ↔ DIN 125-2 A A 3,2:57
- Mate:175: COTS_HP_BLC7000_Fan_Case:1 ↔ DIN 125-2 A A 3,2:59
- Mate:176: COTS_HP_BLC7000_Fan_Case:1 ↔ DIN 125-2 A A 3,2:59
- Insert:61: ISO 7380-1 M3 x 30:1 ↔ DIN 125-2 A A 3,2:57
- Insert:62: ISO 7380-1 M3 x 30:2 ↔ DIN 125-2 A A 3,2:59
- Mate:177: COTS_HP_BLC7000_Fan_Case:1 ↔ DIN 125-2 A A 3,2:58
- Mate:178: 3DP_PLA_Filter_stage_to_turbine_adapter:1 ↔ DIN 125-2 A A 3,2:58
- Mate:179: COTS_HP_BLC7000_Fan_Case:1 ↔ DIN 125-2 A A 3,2:60
- Mate:180: 3DP_PLA_Filter_stage_to_turbine_adapter:1 ↔ DIN 125-2 A A 3,2:60
- Insert:63: DIN 934 - replaced by DIN EN 24032/28673/28674 M3:29 ↔ DIN 125-2 A A 3,2:58
- Insert:64: DIN 934 - replaced by DIN EN 24032/28673/28674 M3:30 ↔ DIN 125-2 A A 3,2:60
- Mate:181: COTS_HP_BLC7000_Fan_Case:1 ↔ DIN 125-2 A A 3,2:61
- Mate:182: COTS_HP_BLC7000_Fan_Case:1 ↔ DIN 125-2 A A 3,2:61
- Mate:183: COTS_HP_BLC7000_Fan_Case:1 ↔ DIN 125-2 A A 3,2:63
- Mate:184: COTS_HP_BLC7000_Fan_Case:1 ↔ DIN 125-2 A A 3,2:63
- Insert:65: ISO 7380-1 M3 x 30:3 ↔ DIN 125-2 A A 3,2:61
- Insert:66: ISO 7380-1 M3 x 30:4 ↔ DIN 125-2 A A 3,2:63
- Mate:185: COTS_HP_BLC7000_Fan_Case:1 ↔ DIN 125-2 A A 3,2:62
- Mate:186: 3DP_PLA_Turbine_exhaust_bottom_part:1 ↔ DIN 125-2 A A 3,2:62
- Mate:187: COTS_HP_BLC7000_Fan_Case:1 ↔ DIN 125-2 A A 3,2:64
- Mate:188: 3DP_PLA_Turbine_exhaust_bottom_part:1 ↔ DIN 125-2 A A 3,2:64
- Insert:67: DIN 934 - replaced by DIN EN 24032/28673/28674 M3:31 ↔ DIN 125-2 A A 3,2:62
- Insert:68: DIN 934 - replaced by DIN EN 24032/28673/28674 M3:32 ↔ DIN 125-2 A A 3,2:64
- Mate:189: 3DP_PLA_Battery_mount:1 ↔ DIN 125-2 A A 4,3:5
- Mate:190: 3DP_PLA_Battery_mount:1 ↔ DIN 125-2 A A 4,3:5
- Mate:191: 3DP_PLA_Battery_mount:2 ↔ DIN 125-2 A A 4,3:7
- Mate:192: 3DP_PLA_Battery_mount:1 ↔ DIN 125-2 A A 4,3:7
- Insert:69: ISO 7380-1 M4 x 20:1 ↔ DIN 125-2 A A 4,3:5
- Insert:70: ISO 7380-1 M4 x 20:2 ↔ DIN 125-2 A A 4,3:7
- Mate:193: 3DP_PLA_Battery_mount:1 ↔ DIN 125-2 A A 4,3:6
- Mate:194: 3DP_PLA_Battery_mount:1 ↔ DIN 125-2 A A 4,3:6
- Mate:195: 3DP_PLA_Battery_mount:2 ↔ DIN 125-2 A A 4,3:8
- Mate:196: 3DP_PLA_Battery_mount:1 ↔ DIN 125-2 A A 4,3:8
- Insert:71: DIN 934 - replaced by DIN EN 24032/28673/28674 M4:3 ↔ DIN 125-2 A A 4,3:6
- Insert:72: DIN 934 - replaced by DIN EN 24032/28673/28674 M4:4 ↔ DIN 125-2 A A 4,3:8
- Mate:197: 3DP_PLA_Switch_&_handle_mount_plate:1 ↔ DIN 125-2 A A 4,3:9
- Mate:198: 3DP_PLA_Switch_&_handle_mount_plate:1 ↔ DIN 125-2 A A 4,3:9
- Mate:199: 3DP_PLA_Switch_&_handle_mount_plate:1 ↔ DIN 125-2 A A 4,3:10
- Mate:200: 3DP_PLA_Switch_&_handle_mount_plate:1 ↔ DIN 125-2 A A 4,3:10
- Insert:73: ISO 7380-1 M4 x 16:1 ↔ DIN 125-2 A A 4,3:9
- Insert:74: ISO 7380-1 M4 x 16:2 ↔ DIN 125-2 A A 4,3:10
